# Autodesk Inventor assembly: Arms-with-motor
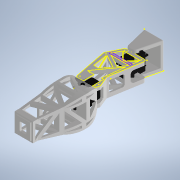
[picture p0: Inventor's stored thumbnail of the model, 180x180]
Saved by Autodesk Inventor 2022 (Build 260153000, 153)
## iProperties
Created: 2022-04-26
Part Number: Arms-with-motor
Document SubType Name: Assembly
Designer: dirks
Author: dirks
## Documents named in this file (6)
- C:\Users\kajve\OneDrive\Documenten\GitHub\Arny-de-humanoid-robot\Parts\Tests\Arms-with-motor.iam
- C:\Users\kajve\OneDrive\Documenten\GitHub\Arny-de-humanoid-robot\Parts\Onderarm(en).ipt
- C:\Users\kajve\OneDrive\Documenten\GitHub\Arny-de-humanoid-robot\Parts\Upper-Arm.ipt
- C:\Users\kajve\OneDrive\Documenten\GitHub\Arny-de-humanoid-robot\Parts\Imported Components\SERVO motor\Servo MOtor.ipt
- C:\Users\kajve\OneDrive\Documenten\GitHub\Arny-de-humanoid-robot\Parts\Imported Components\SERVO motor\Axel Mount.ipt
- C:\Users\kajve\OneDrive\Documenten\GitHub\Arny-de-humanoid-robot\Parts\schouder(s).ipt
## Components (6 placed, 5 different names)
1. Onderarm(en):1 — Mate:5
2. Upper-Arm:1 — Mate:2, Mate:1, Mate:3
3. Servo MOtor:1 — Mate:2, Mate:1, Mate:3, Mate:5
4. Axel Mount:1
5. Servo MOtor:2
6. schouder(s):1
## Relationships (4: Mate 4)
- Mate:2: Upper-Arm:1 ↔ Servo MOtor:1
- Mate:1: Upper-Arm:1 ↔ Servo MOtor:1
- Mate:3 (0.2 mm): Upper-Arm:1 ↔ Servo MOtor:1
- Mate:5 (60 mm): Onderarm(en):1 ↔ Servo MOtor:1
